# Autodesk Inventor assembly: piston_assembled
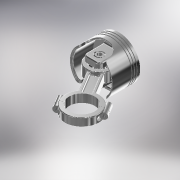
[picture p0: Inventor's stored thumbnail of the model, 180x180]
Saved by Autodesk Inventor 2019 (Build 230136000, 136)
## iProperties
Created: 2020-05-28
Part Number: piston_assembled
Document SubType Name: Assembly
Designer: Manoj
Author: Manoj
## Documents named in this file (5)
- F:\Softwares\Autodesk\YOUTUBE\TotUMentors\piston_assembled.iam
- F:\Softwares\Autodesk\YOUTUBE\TotUMentors\Piston hand.ipt
- F:\Softwares\Autodesk\YOUTUBE\TotUMentors\Piston head.ipt
- F:\Softwares\Autodesk\YOUTUBE\TotUMentors\Piston pin.ipt
- F:\Softwares\Autodesk\YOUTUBE\TotUMentors\Pistonhandattacher.ipt
## Components (4 placed, 4 different names)
1. Piston hand:1 — Mate:1, Mate:2, Mate:3, Flush:1, Mate:4
2. Piston head:1 — Mate:1, Mate:2, Mate:5, Flush:2
3. Piston pin:1 — Mate:5, Flush:2
4. Pistonhandattacher:1 — Mate:3, Flush:1, Mate:4
## Relationships (7: Mate 5, Flush 2)
- Mate:1: Piston hand:1 ↔ Piston head:1
- Mate:2: Piston hand:1 ↔ Piston head:1
- Mate:3: Piston hand:1 ↔ Pistonhandattacher:1
- Flush:1: Piston hand:1 ↔ Pistonhandattacher:1
- Mate:4: Piston hand:1 ↔ Pistonhandattacher:1
- Mate:5: Piston head:1 ↔ Piston pin:1
- Flush:2: Piston head:1 ↔ Piston pin:1
